# Autodesk Inventor assembly: Lifter
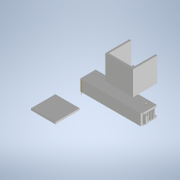
[picture p0: Inventor's stored thumbnail of the model, 180x180]
Saved by Autodesk Inventor 2020 (Build 240168000, 168)
## iProperties
Created: 2021-01-31
Part Number: Lifter
Document SubType Name: Assembly
Designer: moham
Author: moham
## Documents named in this file (5)
- D:\Projects\MCT 131\The project\Lifter\Lifter.iam
- D:\Projects\MCT 131\The project\Lifter\Rack and pinion.iam
- D:\Projects\MCT 131\The project\Lifter\Frontandback_1.ipt
- D:\Projects\MCT 131\The project\Lifter\Sides_2.ipt
- D:\Projects\MCT 131\The project\Lifter\Upperlifter_5.ipt
## Components (12 placed, 4 different names)
1. Rack and pinion:1 [sub-assembly] — Mate:1, Flush:1, Flush:2, Flush:3, Flush:4, Mate:2
2. Rack and pinion:2 [sub-assembly] — Mate:1, Flush:1, Flush:2, Mate:3, Flush:5, Flush:6, Mate:4
3. Rack and pinion:3 [sub-assembly] — Flush:3, Flush:4, Mate:2
4. Rack and pinion:4 [sub-assembly] — Mate:3, Flush:5, Flush:6, Flush:8, Flush:12
5. Frontandback_1:1 — Mate:4, Flush:8, Flush:9, Mate:5, Flush:10, Mate:6, Mate:7, Flush:11, Flush:12
6. Sides_2:1 — Flush:9, Mate:5, Flush:10
7. Sides_2:2 — Mate:6, Mate:7, Flush:11
8. Upperlifter_5:1 — Flush:19, Mate:11, Flush:20
9. Upperlifter_5:2 — Mate:9, Flush:16, Mate:10, Flush:18, Flush:19, Mate:11
10. Upperlifter_5:3 — Mate:9, Flush:16, Flush:17, Flush:20
11. Upperlifter_5:4 — Mate:10, Flush:17, Flush:18
12. Upperlifter_5:5
## Relationships (26: Flush 16, Mate 10)
- Mate:1: Rack and pinion:1 ↔ Rack and pinion:2
- Flush:1: Rack and pinion:1 ↔ Rack and pinion:2
- Flush:2: Rack and pinion:1 ↔ Rack and pinion:2
- Flush:3: Rack and pinion:1 ↔ Rack and pinion:3
- Flush:4: Rack and pinion:1 ↔ Rack and pinion:3
- Mate:2: Rack and pinion:1 ↔ Rack and pinion:3
- Mate:3: Rack and pinion:2 ↔ Rack and pinion:4
- Flush:5: Rack and pinion:2 ↔ Rack and pinion:4
- Flush:6: Rack and pinion:2 ↔ Rack and pinion:4
- Mate:4: Rack and pinion:2 ↔ Frontandback_1:1
- Flush:8 (-0.5 mm): Rack and pinion:4 ↔ Frontandback_1:1
- Flush:9: Frontandback_1:1 ↔ Sides_2:1
- Mate:5: Frontandback_1:1 ↔ Sides_2:1
- Flush:10: Frontandback_1:1 ↔ Sides_2:1
- Mate:6: Frontandback_1:1 ↔ Sides_2:2
- Mate:7: Frontandback_1:1 ↔ Sides_2:2
- Flush:11: Frontandback_1:1 ↔ Sides_2:2
- Flush:12: Rack and pinion:4 ↔ Frontandback_1:1
- Mate:9: Upperlifter_5:2 ↔ Upperlifter_5:3
- Flush:16: Upperlifter_5:2 ↔ Upperlifter_5:3
- Mate:10: Upperlifter_5:2 ↔ Upperlifter_5:4
- Flush:17: Upperlifter_5:3 ↔ Upperlifter_5:4
- Flush:18: Upperlifter_5:2 ↔ Upperlifter_5:4
- Flush:19: Upperlifter_5:1 ↔ Upperlifter_5:2
- Mate:11: Upperlifter_5:1 ↔ Upperlifter_5:2
- Flush:20: Upperlifter_5:1 ↔ Upperlifter_5:3
